# Autodesk Inventor assembly: Mold_h
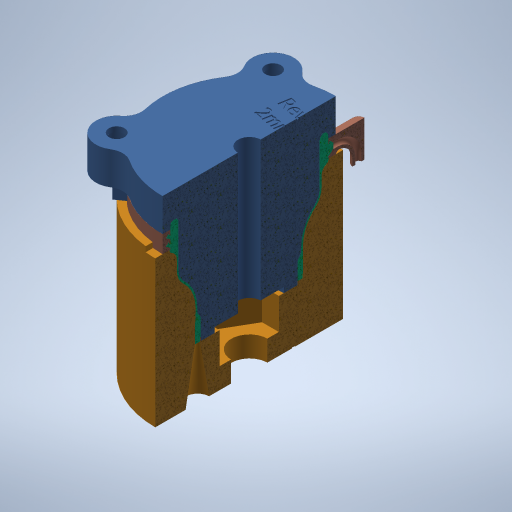
[picture p0: Inventor's stored thumbnail of the model, 512x512]
Saved by Autodesk Inventor 2023.3 (Build 273359000, 359)
## iProperties
Created: 2022-12-01
Part Number: Mold_h
Document SubType Name: Assembly
Designer: splath
Author: splath
## Documents named in this file (5)
- C:\Users\ak-stelzer\source\repos\artgolden\light_sheet_specimen_chambers\Flexible seal for high NA objectives\Mold_and_seal_assembly\Mold_h.iam
- C:\Users\ak-stelzer\source\repos\artgolden\light_sheet_specimen_chambers\Flexible seal for high NA objectives\Mold_and_seal_assembly\Mold_2_Sealing_ring_20x1_silicone_h.ipt
- C:\Users\ak-stelzer\source\repos\artgolden\light_sheet_specimen_chambers\Flexible seal for high NA objectives\Mold_and_seal_assembly\Sealing_ring_20x1_silicone_i.ipt
- C:\Users\ak-stelzer\source\repos\artgolden\light_sheet_specimen_chambers\Flexible seal for high NA objectives\Mold_and_seal_assembly\Mold_1_Sealing_ring_20x1_silicone_x.ipt
- C:\Users\ak-stelzer\source\repos\artgolden\light_sheet_specimen_chambers\Flexible seal for high NA objectives\Mold_and_seal_assembly\Sealing_silicone_i.ipt
## Components (4 placed, 4 different names)
1. Mold_1_Sealing_ring_20x1_silicone_x:2 — Rotational:1
2. Mold_2_Sealing_ring_20x1_silicone_h:1
3. Sealing_ring_20x1_silicone_i:1
4. Sealing_silicone_i:1 — Rotational:1
## Relationships (1: RevoluteJoint 1)
- Rotational:1 [RevoluteJoint]: Mold_1_Sealing_ring_20x1_silicone_x:2 ↔ Sealing_silicone_i:1
